# Autodesk Inventor assembly: volume
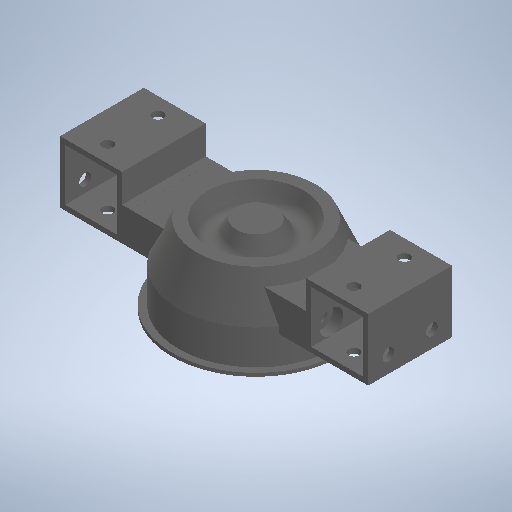
[picture p0: Inventor's stored thumbnail of the model, 512x512]
Saved by Autodesk Inventor 2026.1 (Build 301233020, 233B)
## iProperties
Created: 2026-02-01
Part Number: volume
Document SubType Name: Assembly
Designer: hibik
Author: hibik
## Documents named in this file (3)
- C:\Users\hibik\Documents\Robomech\HR\controller\hard\body\volume.iam
- C:\Users\hibik\Documents\Robomech\HR\controller\hard\body\volume_handle.ipt
- C:\Users\hibik\Documents\Robomech\HR\controller\hard\body\pole_setter.ipt
## Components (3 placed, 2 different names)
1. volume_handle:1 — 挿入:5, 角度:4, 挿入:6, 角度:6, フラッシュ:1, フラッシュ:2, フラッシュ:3
2. pole_setter:2 — 挿入:5, 角度:4
3. pole_setter:4 — 挿入:6, 角度:6
## Relationships (7: Flush 3, Insert 2, Angle 2)
- 挿入:5 [Insert]: volume_handle:1 ↔ pole_setter:2
- 角度:4 [Angle] (0 deg): volume_handle:1 ↔ pole_setter:2
- 挿入:6 [Insert]: volume_handle:1 ↔ pole_setter:4
- 角度:6 [Angle] (0 deg): volume_handle:1 ↔ pole_setter:4
- フラッシュ:1 [Flush]: volume_handle:1
- フラッシュ:2 [Flush]: volume_handle:1
- フラッシュ:3 [Flush]: volume_handle:1
